# Autodesk Inventor assembly: Assiemepinza
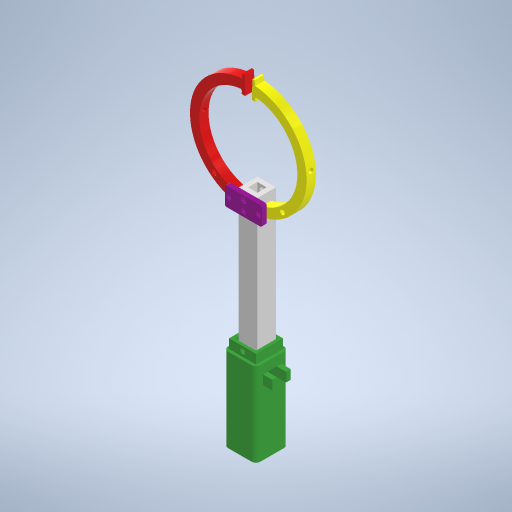
[picture p0: Inventor's stored thumbnail of the model, 512x512]
Saved by Autodesk Inventor 2023 (Build 270158000, 158)
## iProperties
Created: 2023-08-01
Part Number: Assiemepinza
Document SubType Name: Assembly
Designer: Admin
Author: Admin
## Documents named in this file (5)
- C:\Users\Admin\Desktop\3DDDD\da stampanre\08-01-2023 pezzi per pinza telescopica\Assiemepinza.iam
- C:\Users\Admin\Desktop\3DDDD\da stampanre\08-01-2023 pezzi per pinza telescopica\asta.ipt
- C:\Users\Admin\Desktop\3DDDD\da stampanre\08-01-2023 pezzi per pinza telescopica\ganascia.ipt
- C:\Users\Admin\Desktop\3DDDD\da stampanre\08-01-2023 pezzi per pinza telescopica\manico.ipt
- C:\Users\Admin\Desktop\3DDDD\da stampanre\08-01-2023 pezzi per pinza telescopica\perno.ipt
## Components (5 placed, 4 different names)
1. asta:1 — Coincidente:5, Coincidente:6, Coincidente:7, Coincidente:8
2. ganascia:1 — Coincidente:9, Coincidente:11, Coincidente:13
3. ganascia:2 — Coincidente:10, Coincidente:12, Coincidente:13
4. manico:1 — Coincidente:5
5. perno:1 — Coincidente:6, Coincidente:7, Coincidente:8, Coincidente:9, Coincidente:10, Coincidente:11, Coincidente:12
## Relationships (9: Mate 9)
- Coincidente:5 [Mate]: asta:1 ↔ manico:1
- Coincidente:6 [Mate]: asta:1 ↔ perno:1
- Coincidente:7 [Mate]: asta:1 ↔ perno:1
- Coincidente:8 [Mate]: asta:1 ↔ perno:1
- Coincidente:9 [Mate]: ganascia:1 ↔ perno:1
- Coincidente:10 [Mate]: ganascia:2 ↔ perno:1
- Coincidente:11 [Mate]: ganascia:1 ↔ perno:1
- Coincidente:12 [Mate]: ganascia:2 ↔ perno:1
- Coincidente:13 [Mate]: ganascia:1 ↔ ganascia:2
